# Autodesk Inventor assembly: Camera
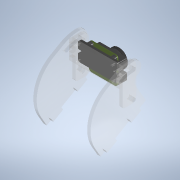
[picture p0: Inventor's stored thumbnail of the model, 180x180]
Saved by Autodesk Inventor 2020 (Build 240168000, 168)
## iProperties
Created: 2019-08-05
Part Number: Camera
Document SubType Name: Assembly
Designer: n10208577
Author: n10208577
## Documents named in this file (8)
- C:\Users\n10208577\Desktop\DRC\DRC2020-Hardware\Design\Camera.iam
- C:\Users\n10208577\Desktop\DRC\DRC2020-Hardware\Design\lense.ipt
- C:\Users\n10208577\Desktop\DRC\DRC2020-Hardware\Design\rpiCam.ipt
- C:\Users\n10208577\Desktop\DRC\DRC2020-Hardware\Design\rpiCamM12Mount.ipt
- C:\Users\n10208577\Desktop\DRC\DRC2020-Hardware\Design\rpiCamMount.ipt
- C:\Users\n10208577\Desktop\DRC\DRC2020-Hardware\Design\camMountBacking.ipt
- C:\Users\n10208577\Desktop\DRC\DRC2020-Hardware\Design\camMountBracket.ipt
- C:\Users\n10208577\Desktop\DRC\DRC2020-Hardware\Design\camMount.ipt
## Components (9 placed, 7 different names)
1. lense:1 — Insert:3
2. rpiCam:1 — Insert:1, Insert:2, Insert:4, Insert:5
3. rpiCamM12Mount:1 — Insert:1, Insert:2, Insert:3
4. rpiCamMount:1 — Insert:4, Insert:5, Insert:6, Insert:7
5. camMountBacking:1 — Insert:6, Insert:7, Mate:1, Mate:2, Mate:3, Mate:4
6. camMountBracket:1 — Mate:1, Mate:2, Insert:8, Angle:2
7. camMountBracket:2 — Mate:3, Mate:4, Insert:9
8. camMount:1 — Insert:8, Angle:1, Angle:2, Angle:3
9. camMount:2 — Insert:9, Angle:1, Angle:3
## Relationships (16: Insert 9, Mate 4, Angle 3)
- Insert:1: rpiCam:1 ↔ rpiCamM12Mount:1
- Insert:2: rpiCam:1 ↔ rpiCamM12Mount:1
- Insert:3: lense:1 ↔ rpiCamM12Mount:1
- Insert:4: rpiCam:1 ↔ rpiCamMount:1
- Insert:5: rpiCam:1 ↔ rpiCamMount:1
- Insert:6: rpiCamMount:1 ↔ camMountBacking:1
- Insert:7: rpiCamMount:1 ↔ camMountBacking:1
- Mate:1: camMountBacking:1 ↔ camMountBracket:1
- Mate:2: camMountBacking:1 ↔ camMountBracket:1
- Mate:3: camMountBacking:1 ↔ camMountBracket:2
- Mate:4: camMountBacking:1 ↔ camMountBracket:2
- Insert:8: camMountBracket:1 ↔ camMount:1
- Insert:9: camMountBracket:2 ↔ camMount:2
- Angle:1 (0 deg): camMount:1 ↔ camMount:2
- Angle:2 (30 deg): camMountBracket:1 ↔ camMount:1
- Angle:3 (0 deg): camMount:1 ↔ camMount:2
